# Autodesk Inventor assembly: beetle
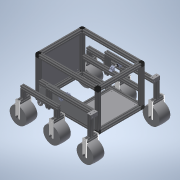
[picture p0: Inventor's stored thumbnail of the model, 180x180]
Saved by Autodesk Inventor 2021 (Build 250183000, 183)
## iProperties
Created: 2021-07-09
Part Number: beetle
Material: 一般
Document SubType Name: Assembly
Designer: gisen
Mass: 47360.5 g
Surface Area: 66475.9 cm^2
Volume: 35407.1 cm^3
Density: 1.3376 g/cm^3
Author: gisen
## Documents named in this file (4)
- C:\Users\gisen\workspace\beetle_inventor_model\beetle.iam
- C:\Users\gisen\workspace\beetle_inventor_model\body\body.iam
- C:\Users\gisen\workspace\beetle_inventor_model\suspension\rocker_bogie_left.iam
- C:\Users\gisen\workspace\beetle_inventor_model\suspension\rocker_bogie_right.iam
## Components (3 placed, 3 different names)
1. body:1 [sub-assembly] — フラッシュ:1, フラッシュ:2, メイト:2, メイト:3, メイト:4, メイト:6, メイト:7
2. rocker_bogie_left:1 [sub-assembly] — メイト:1, メイト:2, メイト:3, メイト:7
3. rocker_bogie_right:1 [sub-assembly] — メイト:4, メイト:5, メイト:6
## Relationships (9: Mate 7, Flush 2)
- フラッシュ:1 [Flush]: body:1
- フラッシュ:2 [Flush]: body:1
- メイト:1 [Mate]: rocker_bogie_left:1
- メイト:2 [Mate]: body:1 ↔ rocker_bogie_left:1
- メイト:3 [Mate]: body:1 ↔ rocker_bogie_left:1
- メイト:4 [Mate]: body:1 ↔ rocker_bogie_right:1
- メイト:5 [Mate]: rocker_bogie_right:1
- メイト:6 [Mate]: body:1 ↔ rocker_bogie_right:1
- メイト:7 [Mate]: body:1 ↔ rocker_bogie_left:1
